# Autodesk Inventor assembly: Claw7
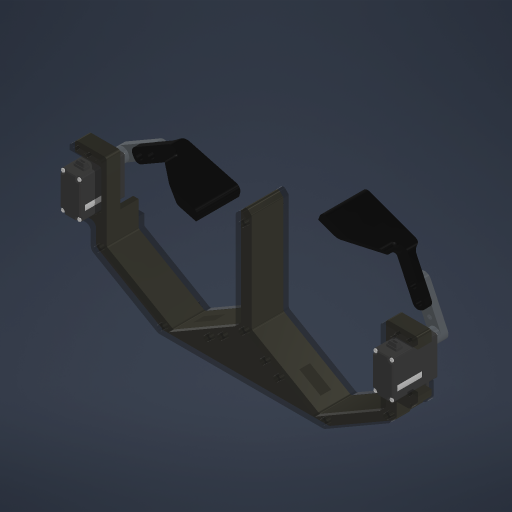
[picture p0: Inventor's stored thumbnail of the model, 512x512]
Saved by Autodesk Inventor 2023 (Build 270158000, 158)
## iProperties
Created: 2023-12-30
Part Number: Claw7
Document SubType Name: Assembly
Designer: kelle
Author: kelle
## Documents named in this file (10)
- C:\Users\kelle\OneDrive\Documents\ENDEAVOR\Claw7.iam
- C:\Users\kelle\OneDrive\Documents\ENDEAVOR\Claw7_Base.ipt
- C:\Users\kelle\OneDrive\Documents\ENDEAVOR\Claw7_Top_Plate.ipt
- C:\Users\kelle\OneDrive\Documents\ENDEAVOR\Claw7_Bottom_Plate.ipt
- C:\Users\kelle\OneDrive\Documents\ENDEAVOR\Raw Files\Axon_MICRO.ipt
- C:\Users\kelle\OneDrive\Documents\ENDEAVOR\Raw Files\Axon_MICRO_MIR2.ipt
- C:\Users\kelle\OneDrive\Documents\ENDEAVOR\Raw Files\Axon_Servo_Arm.ipt
- C:\Users\kelle\OneDrive\Documents\ENDEAVOR\Raw Files\Axon_Servo_Arm_MIR2.ipt
- C:\Users\kelle\OneDrive\Documents\New_Servo_Arms.ipt
- C:\Users\kelle\OneDrive\Documents\New_Servo_Arms_MIR.ipt
## Components (9 placed, 9 different names)
1. Claw7_Base:1 — Mate:3, Mate:4, Angle:2, Mate:5, Angle:5, Angle:6, Mate:6, Mate:7
2. Claw7_Top_Plate:1 — Mate:7
3. Claw7_Bottom_Plate:1 — Mate:3, Mate:4
4. Axon_MICRO:1 — Angle:2, Mate:5, Insert:3
5. Axon_MICRO_MIR2:1 — Insert:2, Angle:6, Mate:6
6. Axon_Servo_Arm:1 — Insert:3, Angle:7, Mate:10
7. Axon_Servo_Arm_MIR2:1 — Angle:5, Insert:2, Mate:9
8. New_Servo_Arms:1 — Angle:7, Mate:10
9. New_Servo_Arms_MIR:1 — Mate:9
## Relationships (13: Mate 7, Angle 4, Insert 2)
- Mate:3: Claw7_Base:1 ↔ Claw7_Bottom_Plate:1
- Mate:4: Claw7_Base:1 ↔ Claw7_Bottom_Plate:1
- Angle:2 (0 deg): Claw7_Base:1 ↔ Axon_MICRO:1
- Mate:5: Claw7_Base:1 ↔ Axon_MICRO:1
- Angle:5 (0 deg): Claw7_Base:1 ↔ Axon_Servo_Arm_MIR2:1
- Insert:2: Axon_MICRO_MIR2:1 ↔ Axon_Servo_Arm_MIR2:1
- Angle:6 (0 deg): Claw7_Base:1 ↔ Axon_MICRO_MIR2:1
- Mate:6: Claw7_Base:1 ↔ Axon_MICRO_MIR2:1
- Mate:7: Claw7_Base:1 ↔ Claw7_Top_Plate:1
- Mate:9: Axon_Servo_Arm_MIR2:1 ↔ New_Servo_Arms_MIR:1
- Insert:3: Axon_MICRO:1 ↔ Axon_Servo_Arm:1
- Angle:7 (0 deg): Axon_Servo_Arm:1 ↔ New_Servo_Arms:1
- Mate:10: Axon_Servo_Arm:1 ↔ New_Servo_Arms:1
